# Autodesk Inventor assembly: POM_T5_04
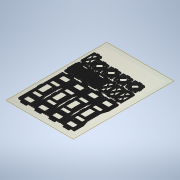
[picture p0: Inventor's stored thumbnail of the model, 180x180]
Saved by Autodesk Inventor 2020 (Build 240168000, 168)
## iProperties
Created: 2021-08-27
Part Number: POM_T5_04
Document SubType Name: Assembly
Designer: Masato
Author: Masato
## Documents named in this file (6)
- C:\Users\L20C1118 森　圭汰\Documents\20220327_open\SUSTAINA-OP\Cam\POM_T5_04.iam
- C:\Users\L20C1118 森　圭汰\Documents\20220327_open\SUSTAINA-OP\Cam\DisposableBoard.ipt
- C:\Users\L20C1118 森　圭汰\Documents\20220327_open\SUSTAINA-OP\UpperBody\Trunk\Trunk_chest_frame.ipt
- C:\Users\L20C1118 森　圭汰\Documents\20220327_open\SUSTAINA-OP\UpperBody\Head\Camera_root_frame.ipt
- C:\Users\L20C1118 森　圭汰\Documents\20220327_open\SUSTAINA-OP\UpperBody\Head\Head_diagonal.ipt
- C:\Users\L20C1118 森　圭汰\Documents\20220327_open\SUSTAINA-OP\UpperBody\Arm\UpperArm_diagonal.ipt
## Components (15 placed, 5 different names)
1. DisposableBoard:1 — メイト:2, メイト:1, フラッシュ:1, フラッシュ:2, メイト:5, メイト:7, メイト:9, メイト:11, メイト:13, フラッシュ:9, フラッシュ:10
2. Head_diagonal:4 — メイト:9, フラッシュ:7, メイト:10, フラッシュ:8, メイト:12
3. Camera_root_frame:1 — メイト:5, フラッシュ:7, メイト:10, メイト:14, フラッシュ:11
4. Camera_root_frame:2 — フラッシュ:6, メイト:8
5. Head_diagonal:1 — メイト:7, フラッシュ:6, メイト:8
6. Head_diagonal:2
7. Head_diagonal:3
8. UpperArm_diagonal:1 — メイト:11, フラッシュ:8, メイト:12
9. UpperArm_diagonal:2
10. UpperArm_diagonal:3
11. UpperArm_diagonal:4
12. Trunk_chest_frame:1 — メイト:13, フラッシュ:9, フラッシュ:10, メイト:14, フラッシュ:11
13. Trunk_chest_frame:2
14. Trunk_chest_frame:3
15. Trunk_chest_frame:4
## Component patterns: (2 elements, first: Camera_root_frame:1), (3 elements, first: Head_diagonal:1), (4 elements, first: UpperArm_diagonal:1), (4 elements, first: Trunk_chest_frame:1)
## Relationships (19: Mate 11, Flush 8)
- メイト:2 [Mate]: DisposableBoard:1
- メイト:1 [Mate]: DisposableBoard:1
- フラッシュ:1 [Flush]: DisposableBoard:1
- フラッシュ:2 [Flush]: DisposableBoard:1
- メイト:5 [Mate]: DisposableBoard:1 ↔ Camera_root_frame:1
- メイト:7 [Mate]: DisposableBoard:1 ↔ Head_diagonal:1
- フラッシュ:6 [Flush]: Camera_root_frame:2 ↔ Head_diagonal:1
- メイト:8 [Mate] (2.5 mm): Camera_root_frame:2 ↔ Head_diagonal:1
- メイト:9 [Mate]: DisposableBoard:1 ↔ Head_diagonal:4
- フラッシュ:7 [Flush]: Head_diagonal:4 ↔ Camera_root_frame:1
- メイト:10 [Mate] (2.5 mm): Head_diagonal:4 ↔ Camera_root_frame:1
- メイト:11 [Mate]: DisposableBoard:1 ↔ UpperArm_diagonal:1
- フラッシュ:8 [Flush]: Head_diagonal:4 ↔ UpperArm_diagonal:1
- メイト:12 [Mate] (2.5 mm): Head_diagonal:4 ↔ UpperArm_diagonal:1
- メイト:13 [Mate]: DisposableBoard:1 ↔ Trunk_chest_frame:1
- フラッシュ:9 [Flush] (2.5 mm): DisposableBoard:1 ↔ Trunk_chest_frame:1
- フラッシュ:10 [Flush] (-2.5 mm): DisposableBoard:1 ↔ Trunk_chest_frame:1
- メイト:14 [Mate] (2.5 mm): Camera_root_frame:1 ↔ Trunk_chest_frame:1
- フラッシュ:11 [Flush]: Camera_root_frame:1 ↔ Trunk_chest_frame:1
